# Autodesk Inventor assembly: Z Assembly
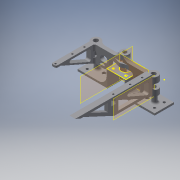
[picture p0: Inventor's stored thumbnail of the model, 180x180]
Saved by Autodesk Inventor 2016 (Build 200138000, 138)
## iProperties
Created: 2014-11-03
Part Number: Z Assembly
Document SubType Name: Assembly
Designer: Scott
Author: Scott
## Documents named in this file (4)
- C:\Users\Scott\Google Drive\Engineering Ideas and Designs\3D printer\PISCES\Parts\Z Assembly.iam
- C:\Users\Scott\Google Drive\Engineering Ideas and Designs\3D printer\PISCES\Parts\Base plate.ipt
- C:\Users\Scott\Google Drive\Engineering Ideas and Designs\3D printer\PISCES\Parts\Plate Carrier.ipt
- C:\Users\Scott\Google Drive\Engineering Ideas and Designs\3D printer\PISCES\Parts\PlateSpacer.ipt
## Components (3 placed, 3 different names)
1. Base plate:1
2. Plate Carrier:1 — Flush:1, Flush:2, Flush:3
3. PlateSpacer:1 — Flush:1, Flush:2, Flush:3
## Relationships (3: Flush 3)
- Flush:1: Plate Carrier:1 ↔ PlateSpacer:1
- Flush:2: Plate Carrier:1 ↔ PlateSpacer:1
- Flush:3: Plate Carrier:1 ↔ PlateSpacer:1
